# Autodesk Inventor assembly: ASSY_REV,ENG_DESIGN2
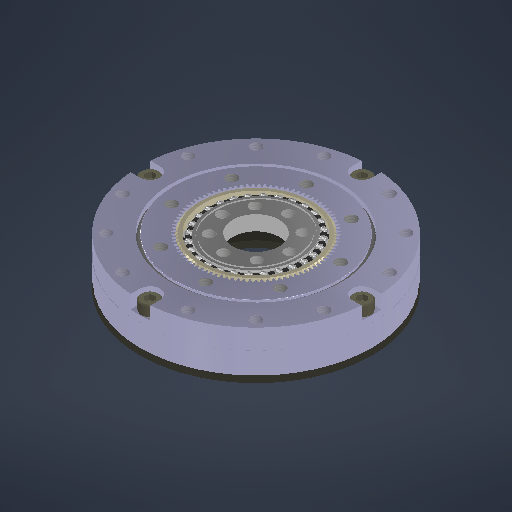
[picture p0: Inventor's stored thumbnail of the model, 512x512]
Saved by Autodesk Inventor 2026.2 (Build 302298010, 298A)
## iProperties
Created: 2026-02-10
Part Number: ASSY_REV,ENG_DESIGN2
Document SubType Name: Assembly
Designer: 4aida
Author: 4aida
## Documents named in this file (16)
- C:\Users\4aida\OneDrive\Documents\GitHub\Design_II_Group6\REV_ENG\ASSY_REV,ENG_DESIGN2.iam
- C:\Users\4aida\OneDrive\Documents\GitHub\Design_II_Group6\REV_ENG\ROLLER_CR_BEARING,REV-ENG.ipt
- C:\Users\4aida\OneDrive\Documents\GitHub\Design_II_Group6\REV_ENG\SPACER_ROLLER_CR_BEARING,REV-ENG.ipt
- C:\Users\4aida\OneDrive\Documents\GitHub\Design_II_Group6\REV_ENG\MIR_SPACER_ROLLER_CR_BEARING,REV-ENG.ipt
- C:\Users\4aida\OneDrive\Documents\GitHub\Design_II_Group6\REV_ENG\CR_ROLLER_BOUNDRY,REV-ENG.ipt
- C:\Users\4aida\OneDrive\Documents\GitHub\Design_II_Group6\REV_ENG\O_RING.ipt
- C:\Users\4aida\OneDrive\Documents\GitHub\Design_II_Group6\REV_ENG\CR_OUTSIDE,BOTTOM,REV-ENG.ipt
- C:\Users\4aida\OneDrive\Documents\GitHub\Design_II_Group6\REV_ENG\CR_OUTSIDE,TOP,REV-ENG.ipt
- C:\Users\4aida\OneDrive\Documents\GitHub\Design_II_Group6\REV_ENG\Fasteners\M3\SCREW,SOCKET-HD,P,12_9,M03X0_5X10MM.ipt
- C:\Users\4aida\OneDrive\Documents\GitHub\Design_II_Group6\REV_ENG\2.5mm_BALL_BEARINGS.ipt
- C:\Users\4aida\OneDrive\Documents\GitHub\Design_II_Group6\REV_ENG\Flex_SPLINE,REV-ENG.iam
- C:\Users\4aida\OneDrive\Documents\GitHub\Design_II_Group6\REV_ENG\DERIVEN_CR_INSIDE,REV-ENG.ipt
- C:\Users\4aida\OneDrive\Documents\GitHub\Design_II_Group6\REV_ENG\ELIPSE_DRIVE,REV-ENG.ipt
- C:\Users\4aida\OneDrive\Documents\GitHub\Design_II_Group6\REV_ENG\BOTTOM_ELIP_BEARING_SEAL,REV-ENG.ipt
- C:\Users\4aida\OneDrive\Documents\GitHub\Design_II_Group6\REV_ENG\DERIVEN_BALL_BEARING,REV-ENG.ipt
- C:\Users\4aida\OneDrive\Documents\GitHub\Design_II_Group6\REV_ENG\STRAIN_WAVE_BASS_PLATE,REV-ENG.ipt
## Components (63 placed, 15 different names)
1. CR_ROLLER_BOUNDRY,REV-ENG:1 — Mate:23, Mate:24
2. O_RING:1 — Mate:16, Tangent:7
3. CR_OUTSIDE,BOTTOM,REV-ENG:1 — Mate:9, Mate:10, Mate:13, Flush:4, Mate:25, Mate:26, Mate:38, Mate:39
4. CR_OUTSIDE,TOP,REV-ENG:1 — Mate:9, Mate:10, Mate:12, Insert:1, Insert:2, Insert:3, Insert:4, Mate:27, Mate:28, Flush:8
5. SCREW,SOCKET-HD,P,12_9,M03X0_5X10MM:1 — Insert:1
6. Flex_SPLINE,REV-ENG:1 [sub-assembly] — Flush:5, Mate:15, Mate:25, Mate:16, Mate:29
7. DERIVEN_CR_INSIDE,REV-ENG:1 — Flush:5, Mate:15, Tangent:7, Mate:18, Mate:21, Tangent:8, Tangent:9, Mate:28, Flush:8, Flush:9, Rotation:1
8. SCREW,SOCKET-HD,P,12_9,M03X0_5X10MM:2 — Insert:4
9. SCREW,SOCKET-HD,P,12_9,M03X0_5X10MM:3 — Insert:2
10. SCREW,SOCKET-HD,P,12_9,M03X0_5X10MM:4 — Insert:3, Mate:40
11. ELIPSE_DRIVE,REV-ENG:1 — Flush:9, Tangent:10, Mate:31, Flush:10, Mate:33, Rotation:1, Mate:34, Mate:35, Mate:37
12. 2.5mm_BALL_BEARINGS:3 — Mate:30, Tangent:10, Mate:31, Mate:36
13. BOTTOM_ELIP_BEARING_SEAL,REV-ENG:1 — Mate:32, Flush:10, Mate:33
14. DERIVEN_BALL_BEARING,REV-ENG:1 — Mate:34, Mate:35, Mate:36
15. STRAIN_WAVE_BASS_PLATE,REV-ENG:1 — Mate:38, Mate:39, Mate:40
16. MIR_SPACER_ROLLER_CR_BEARING,REV-ENG:13 — Mate:21, Mate:22
17. ROLLER_CR_BEARING,REV-ENG:27 — Mate:20, Mate:22, Tangent:8
18. SPACER_ROLLER_CR_BEARING,REV-ENG:13 — Mate:18, Mate:19, Flush:7, Mate:20
19. ROLLER_CR_BEARING,REV-ENG:26 — Mate:19, Tangent:9
20. MIR_SPACER_ROLLER_CR_BEARING,REV-ENG:14
21. ROLLER_CR_BEARING,REV-ENG:28
22. SPACER_ROLLER_CR_BEARING,REV-ENG:14
23. ROLLER_CR_BEARING,REV-ENG:29
24. MIR_SPACER_ROLLER_CR_BEARING,REV-ENG:15
25. ROLLER_CR_BEARING,REV-ENG:30
26. SPACER_ROLLER_CR_BEARING,REV-ENG:15
27. ROLLER_CR_BEARING,REV-ENG:31
28. MIR_SPACER_ROLLER_CR_BEARING,REV-ENG:16
29. ROLLER_CR_BEARING,REV-ENG:32
30. SPACER_ROLLER_CR_BEARING,REV-ENG:16
31. ROLLER_CR_BEARING,REV-ENG:33
32. MIR_SPACER_ROLLER_CR_BEARING,REV-ENG:17
33. ROLLER_CR_BEARING,REV-ENG:34
34. SPACER_ROLLER_CR_BEARING,REV-ENG:17
35. ROLLER_CR_BEARING,REV-ENG:35
36. MIR_SPACER_ROLLER_CR_BEARING,REV-ENG:18
37. ROLLER_CR_BEARING,REV-ENG:36
38. SPACER_ROLLER_CR_BEARING,REV-ENG:18
39. ROLLER_CR_BEARING,REV-ENG:37
40. MIR_SPACER_ROLLER_CR_BEARING,REV-ENG:19
41. ROLLER_CR_BEARING,REV-ENG:38
42. SPACER_ROLLER_CR_BEARING,REV-ENG:19
43. ROLLER_CR_BEARING,REV-ENG:39
44. MIR_SPACER_ROLLER_CR_BEARING,REV-ENG:20
45. ROLLER_CR_BEARING,REV-ENG:40
46. SPACER_ROLLER_CR_BEARING,REV-ENG:20
47. ROLLER_CR_BEARING,REV-ENG:41
48. MIR_SPACER_ROLLER_CR_BEARING,REV-ENG:21
49. ROLLER_CR_BEARING,REV-ENG:42
50. SPACER_ROLLER_CR_BEARING,REV-ENG:21
51. ROLLER_CR_BEARING,REV-ENG:43
52. MIR_SPACER_ROLLER_CR_BEARING,REV-ENG:22
53. ROLLER_CR_BEARING,REV-ENG:44
54. SPACER_ROLLER_CR_BEARING,REV-ENG:22
55. ROLLER_CR_BEARING,REV-ENG:45
56. MIR_SPACER_ROLLER_CR_BEARING,REV-ENG:23
57. ROLLER_CR_BEARING,REV-ENG:46
58. SPACER_ROLLER_CR_BEARING,REV-ENG:23
59. ROLLER_CR_BEARING,REV-ENG:47
60. MIR_SPACER_ROLLER_CR_BEARING,REV-ENG:24
61. ROLLER_CR_BEARING,REV-ENG:48
62. SPACER_ROLLER_CR_BEARING,REV-ENG:24
63. ROLLER_CR_BEARING,REV-ENG:49
## Component patterns: (12 elements, first: MIR_SPACER_ROLLER_CR_BEARING,REV-ENG:13 + ROLLER_CR_BEARING,REV-ENG:27 + SPACER_ROLLER_CR_BEARING,REV-ENG:13 + ROLLER_CR_BEARING,REV-ENG:26)
## Relationships (44: Mate 29, Flush 6, Tangent 4, Insert 4, RelateRotation 1)
- Mate:9: CR_OUTSIDE,BOTTOM,REV-ENG:1 ↔ CR_OUTSIDE,TOP,REV-ENG:1
- Mate:10: CR_OUTSIDE,BOTTOM,REV-ENG:1 ↔ CR_OUTSIDE,TOP,REV-ENG:1
- Mate:12: CR_OUTSIDE,TOP,REV-ENG:1
- Mate:13: CR_OUTSIDE,BOTTOM,REV-ENG:1
- Flush:4: CR_OUTSIDE,BOTTOM,REV-ENG:1
- Flush:5: Flex_SPLINE,REV-ENG:1 ↔ DERIVEN_CR_INSIDE,REV-ENG:1
- Mate:15: Flex_SPLINE,REV-ENG:1 ↔ DERIVEN_CR_INSIDE,REV-ENG:1
- Mate:16: O_RING:1 ↔ Flex_SPLINE,REV-ENG:1
- Tangent:7: O_RING:1 ↔ DERIVEN_CR_INSIDE,REV-ENG:1
- Mate:18: DERIVEN_CR_INSIDE,REV-ENG:1 ↔ SPACER_ROLLER_CR_BEARING,REV-ENG:13
- Mate:19: SPACER_ROLLER_CR_BEARING,REV-ENG:13 ↔ ROLLER_CR_BEARING,REV-ENG:26
- Flush:7: SPACER_ROLLER_CR_BEARING,REV-ENG:13
- Mate:20: ROLLER_CR_BEARING,REV-ENG:27 ↔ SPACER_ROLLER_CR_BEARING,REV-ENG:13
- Mate:21: DERIVEN_CR_INSIDE,REV-ENG:1 ↔ MIR_SPACER_ROLLER_CR_BEARING,REV-ENG:13
- Mate:22: MIR_SPACER_ROLLER_CR_BEARING,REV-ENG:13 ↔ ROLLER_CR_BEARING,REV-ENG:27
- Tangent:8 (0.125 mm): DERIVEN_CR_INSIDE,REV-ENG:1 ↔ ROLLER_CR_BEARING,REV-ENG:27
- Tangent:9 (0.125 mm): DERIVEN_CR_INSIDE,REV-ENG:1 ↔ ROLLER_CR_BEARING,REV-ENG:26
- Mate:23: CR_ROLLER_BOUNDRY,REV-ENG:1
- Mate:24: CR_ROLLER_BOUNDRY,REV-ENG:1
- Mate:25: CR_OUTSIDE,BOTTOM,REV-ENG:1 ↔ Flex_SPLINE,REV-ENG:1
- Insert:1: CR_OUTSIDE,TOP,REV-ENG:1 ↔ SCREW,SOCKET-HD,P,12_9,M03X0_5X10MM:1
- Insert:2: CR_OUTSIDE,TOP,REV-ENG:1 ↔ SCREW,SOCKET-HD,P,12_9,M03X0_5X10MM:3
- Insert:3: CR_OUTSIDE,TOP,REV-ENG:1 ↔ SCREW,SOCKET-HD,P,12_9,M03X0_5X10MM:4
- Insert:4: CR_OUTSIDE,TOP,REV-ENG:1 ↔ SCREW,SOCKET-HD,P,12_9,M03X0_5X10MM:2
- Mate:26: CR_OUTSIDE,BOTTOM,REV-ENG:1
- Mate:27: CR_OUTSIDE,TOP,REV-ENG:1
- Mate:28: CR_OUTSIDE,TOP,REV-ENG:1 ↔ DERIVEN_CR_INSIDE,REV-ENG:1
- Flush:8: CR_OUTSIDE,TOP,REV-ENG:1 ↔ DERIVEN_CR_INSIDE,REV-ENG:1
- Flush:9: DERIVEN_CR_INSIDE,REV-ENG:1 ↔ ELIPSE_DRIVE,REV-ENG:1
- Mate:29: Flex_SPLINE,REV-ENG:1
- Mate:30: 2.5mm_BALL_BEARINGS:3
- Tangent:10: ELIPSE_DRIVE,REV-ENG:1 ↔ 2.5mm_BALL_BEARINGS:3
- Mate:31: ELIPSE_DRIVE,REV-ENG:1 ↔ 2.5mm_BALL_BEARINGS:3
- Mate:32: BOTTOM_ELIP_BEARING_SEAL,REV-ENG:1
- Flush:10 (0.375 mm): ELIPSE_DRIVE,REV-ENG:1 ↔ BOTTOM_ELIP_BEARING_SEAL,REV-ENG:1
- Mate:33: ELIPSE_DRIVE,REV-ENG:1 ↔ BOTTOM_ELIP_BEARING_SEAL,REV-ENG:1
- Rotation:1 [RelateRotation] (0.0116 ul): DERIVEN_CR_INSIDE,REV-ENG:1 ↔ ELIPSE_DRIVE,REV-ENG:1
- Mate:34: ELIPSE_DRIVE,REV-ENG:1 ↔ DERIVEN_BALL_BEARING,REV-ENG:1
- Mate:35: ELIPSE_DRIVE,REV-ENG:1 ↔ DERIVEN_BALL_BEARING,REV-ENG:1
- Mate:36: 2.5mm_BALL_BEARINGS:3 ↔ DERIVEN_BALL_BEARING,REV-ENG:1
- Mate:37: ELIPSE_DRIVE,REV-ENG:1
- Mate:38: CR_OUTSIDE,BOTTOM,REV-ENG:1 ↔ STRAIN_WAVE_BASS_PLATE,REV-ENG:1
- Mate:39: CR_OUTSIDE,BOTTOM,REV-ENG:1 ↔ STRAIN_WAVE_BASS_PLATE,REV-ENG:1
- Mate:40: SCREW,SOCKET-HD,P,12_9,M03X0_5X10MM:4 ↔ STRAIN_WAVE_BASS_PLATE,REV-ENG:1
